# Autodesk Inventor assembly: V2-Output-.5inHex
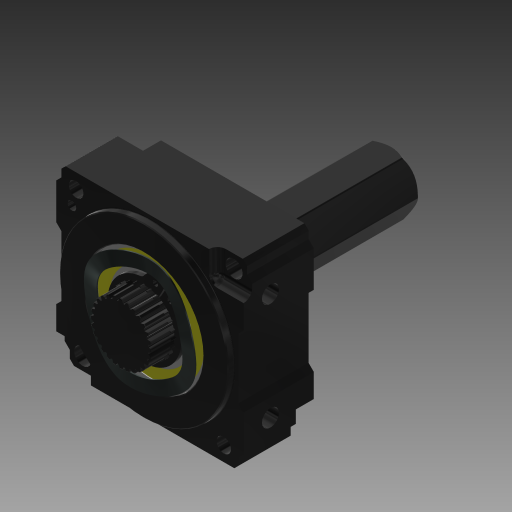
[picture p0: Inventor's stored thumbnail of the model, 512x512]
Saved by Autodesk Inventor 2023 (Build 270158030, 158C)
## iProperties
Created: 2018-08-19
Part Number: V2-Output-.5inHex
Document SubType Name: Assembly
Mass: 68.0389 g
Surface Area: 166.113 cm^2
Volume: 34.5687 cm^3
Density: 1.96822 g/cm^3
## Documents named in this file (8)
- D:\Collaborative Robots\COTS Parts\General Gearboxes\Planetaries\DEPRECATED Versaplanetary\V2 Stages\V2 Output Stage\VP V2 Output Stage 1-2in Hex.iam
- D:\Collaborative Robots\COTS Parts\General Gearboxes\Planetaries\DEPRECATED Versaplanetary\V2 Stages\V2 Output Housing.ipt
- D:\Collaborative Robots\COTS Parts\General Gearboxes\Planetaries\DEPRECATED Versaplanetary\V2 Stages\Wave Washer.ipt
- D:\Collaborative Robots\COTS Parts\General Gearboxes\Planetaries\DEPRECATED Versaplanetary\Output Shafts\VP 1-2inHex Output.ipt
- D:\Collaborative Robots\COTS Parts\General Gearboxes\Planetaries\DEPRECATED Versaplanetary\V2 Stages\Retaining Ring.ipt
- D:\Collaborative Robots\COTS Parts\Power Transfer\Bearings and Bushings\Bearings\6902ZZ.ipt
- E:\Elipse 6814\Elipse Parts Library\Shaft Accessories\Bearings.ipt
- D:\Collaborative Robots\COTS Parts\General Gearboxes\Planetaries\DEPRECATED Versaplanetary\V2 Stages\V2 Output Stage.iam
## Components (6 placed, 5 different names)
1. V2 Output Housing:1 — Insert:2, Mate:2, Insert:18, Mate:3, Angle:6, Flush:7
2. 6902ZZ:1 — Insert:2, Insert:23
3. 6902ZZ:2 — Insert:18, Insert:20
4. Wave Washer:1 — Mate:2
5. Retaining Ring:1 — Angle:1, Insert:23
6. VP 1-2inHex Output:1 — Angle:1, Insert:20
## Relationships (9: Insert 4, Mate 2, Angle 2, Flush 1)
- Insert:2: V2 Output Housing:1 ↔ 6902ZZ:1
- Mate:2: V2 Output Housing:1 ↔ Wave Washer:1
- Angle:1 (0 deg): Retaining Ring:1 ↔ VP 1-2inHex Output:1
- Insert:18: V2 Output Housing:1 ↔ 6902ZZ:2
- Insert:20: 6902ZZ:2 ↔ VP 1-2inHex Output:1
- Insert:23 (0.508 mm): 6902ZZ:1 ↔ Retaining Ring:1
- Mate:3: V2 Output Housing:1
- Angle:6 (0 deg): V2 Output Housing:1
- Flush:7: V2 Output Housing:1
